# Autodesk Inventor assembly: ASM_Micron_Rev_with_Jigs_manipulator
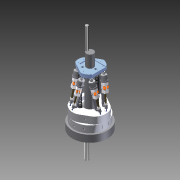
[picture p0: Inventor's stored thumbnail of the model, 180x180]
Saved by Autodesk Inventor 2011 SP2 (Build 150309200, 309)
## iProperties
Created: 2011-09-29
Part Number: ASM_Micron_Rev_with_Jigs_manipulator
Document SubType Name: Assembly
Designer: sungwook
Author: sungwook
## Documents named in this file (6)
- C:\Users\sungwook\Documents\Inventor\Micron20\Assembly\ASM_Micron_Rev_with_Jigs_manipulator.iam
- C:\Users\sungwook\Documents\Inventor\Micron20\Parts\Jigs\Jig_TopHeightAligner.ipt
- C:\Users\sungwook\Documents\Inventor\Micron20\Parts\Jigs\Jig_pin_p080.ipt
- C:\Users\sungwook\Documents\Inventor\Micron20\Parts\Jigs\Jig_pin_p118.ipt
- C:\Users\sungwook\Documents\Inventor\Micron20\Assembly\ASM_Micron_Rev2(manipulator).iam
- C:\Users\sungwook\Documents\Inventor\Micron20\Parts\Jigs\Jig_Aligner_Sleeve.ipt
## Components (5 placed, 5 different names)
1. Jig_TopHeightAligner:1 — Mate:11, Mate:9, Mate:15, Bottom Mate, Mate:20, Mate:21, Mate:22, Mate:23
2. Jig_pin_p080:1 — Mate:11, Mate:16
3. Jig_pin_p118:1 — Mate:9, Mate:17, Mate:18
4. ASM_Micron_Rev2(manipulator):1 [sub-assembly] — Mate:15, Mate:16, Mate:17, Mate:18, Bottom Mate, Mate:20, Mate:23, Mate:24
5. Jig_Aligner_Sleeve:1 — Mate:21, Mate:22, Mate:24
## Relationships (12: Mate 12)
- Mate:9: Jig_TopHeightAligner:1 ↔ Jig_pin_p118:1
- Mate:11: Jig_TopHeightAligner:1 ↔ Jig_pin_p080:1
- Mate:15: Jig_TopHeightAligner:1 ↔ ASM_Micron_Rev2(manipulator):1
- Mate:16: Jig_pin_p080:1 ↔ ASM_Micron_Rev2(manipulator):1
- Mate:17: Jig_pin_p118:1 ↔ ASM_Micron_Rev2(manipulator):1
- Mate:18: Jig_pin_p118:1 ↔ ASM_Micron_Rev2(manipulator):1
- Bottom Mate [Mate]: Jig_TopHeightAligner:1 ↔ ASM_Micron_Rev2(manipulator):1
- Mate:20: Jig_TopHeightAligner:1 ↔ ASM_Micron_Rev2(manipulator):1
- Mate:21: Jig_TopHeightAligner:1 ↔ Jig_Aligner_Sleeve:1
- Mate:22 (0.508 mm): Jig_TopHeightAligner:1 ↔ Jig_Aligner_Sleeve:1
- Mate:23: Jig_TopHeightAligner:1 ↔ ASM_Micron_Rev2(manipulator):1
- Mate:24: ASM_Micron_Rev2(manipulator):1 ↔ Jig_Aligner_Sleeve:1
